# Autodesk Inventor assembly: Gear-Assembly-Draft
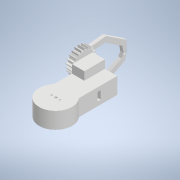
[picture p0: Inventor's stored thumbnail of the model, 180x180]
Saved by Autodesk Inventor 2022 (Build 260153000, 153)
## iProperties
Created: 2022-02-25
Part Number: Gear-Assembly-Draft
Document SubType Name: Assembly
Designer: Alexa
Author: Alexa
## Documents named in this file (4)
- C:\Users\Alexa\Documents\4TH YEAR\ROBOTICS PARTS\NEW PARTS\Gear-Assembly-Draft.iam
- C:\Users\Alexa\Documents\4TH YEAR\ROBOTICS PARTS\NEW PARTS\EndConnector.ipt
- C:\Users\Alexa\Documents\4TH YEAR\ROBOTICS PARTS\NEW PARTS\GearV2-1.ipt
- C:\Users\Alexa\Documents\4TH YEAR\ROBOTICS PARTS\NEW PARTS\GearV2-2.ipt
## Components (3 placed, 3 different names)
1. EndConnector:1 — Rotational:1, Rotational:2
2. GearV2-1:1 — Rotational:1
3. GearV2-2:1 — Rotational:2
## Relationships (2: RevoluteJoint 2)
- Rotational:1 [RevoluteJoint]: EndConnector:1 ↔ GearV2-1:1
- Rotational:2 [RevoluteJoint]: EndConnector:1 ↔ GearV2-2:1
